# Autodesk Inventor assembly: doutai
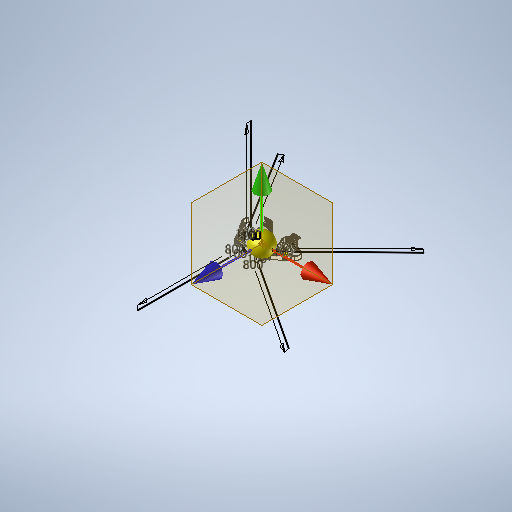
[picture p0: Inventor's stored thumbnail of the model, 512x512]
Saved by Autodesk Inventor 2025.1 (Build 291241000, 241)
## iProperties
Created: 2024-09-01
Part Number: doutai
Document SubType Name: Assembly
Designer: right
Mass: 1092.19 g
Surface Area: 3839.17 cm^2
Volume: 644.209 cm^3
Density: 1.6954 g/cm^3
Author: right
## Documents named in this file (48)
- C:\Users\right\Documents\Inventor\Vixen\doutai.iam
- C:\Users\right\Documents\Inventor\Vixen\KRS2500_scale.ipt
- C:\Users\right\Documents\Inventor\Vixen\02157_SmallDiameterHornB.ipt
- C:\Users\right\Documents\Inventor\Vixen\namida.ipt
- C:\Users\right\Documents\Inventor\Vixen\kataue.ipt
- C:\Users\right\Documents\Inventor\Vixen\kosi_v3_1.5.ipt
- C:\Users\right\Documents\Inventor\Vixen\kosipiti.ipt
- C:\Users\right\Documents\Inventor\Vixen\kosi_pti.ipt
- C:\Users\right\Documents\Inventor\Vixen\suberase.ipt
- C:\Users\right\Documents\Inventor\Vixen\kosipiti - コピー.ipt
- C:\Users\right\Documents\Inventor\Vixen\kosi_pti_MIR.ipt
- C:\Users\right\Documents\Inventor\Vixen\katasita.ipt
- C:\Users\right\Documents\Inventor\Vixen\KSHI.ipt
- C:\Users\right\Documents\Inventor\Vixen\mata3.ipt
- C:\Users\right\Documents\Inventor\Vixen\matasita.ipt
- C:\Users\right\Documents\Inventor\Vixen\kosiuke.ipt
- C:\Users\right\Documents\Inventor\Vixen\02159_SmallFreeHornC\02159_SmallFreeHornC.ipt
- C:\Users\right\Documents\Inventor\Vixen\mataroll.ipt
- C:\Users\right\Documents\Inventor\Vixen\matat3.ipt
- C:\Users\right\Documents\Inventor\Vixen\momo.ipt
- C:\Users\right\Documents\Inventor\Vixen\servolink.ipt
- C:\Users\right\Documents\Inventor\Vixen\free_link.ipt
- C:\Users\right\Documents\Inventor\Vixen\free_suzikai.ipt
- C:\Users\right\Documents\Inventor\Vixen\hiza.ipt
- C:\Users\right\Documents\Inventor\Vixen\fox.ipt
- C:\Users\right\Documents\Inventor\Vixen\mune_1.ipt
- C:\Users\right\Documents\Inventor\Vixen\mune_2.ipt
- C:\Users\right\Documents\Inventor\Vixen\badcase.ipt
- C:\Users\right\Documents\Inventor\Vixen\bad_huta.ipt
- C:\Users\right\Documents\Inventor\Vixen\450mah.ipt
- C:\Users\right\Documents\Inventor\Vixen\asikubi_asi.ipt
- C:\Users\right\Documents\Inventor\Vixen\asikubi_asi_MIR.ipt
- C:\Users\right\Documents\Inventor\Vixen\kata.ipt
- C:\Users\right\Documents\Inventor\Vixen\t3kata.ipt
- C:\Users\right\Documents\Inventor\Vixen\ude.ipt
- C:\Users\right\Documents\Inventor\V2二足Light＿仮\02159_SmallFreeHornC_MIR2.ipt
- C:\Users\right\Documents\Inventor\V2二足Light＿仮\02157_SmallDiameterHornB_MIR1.ipt
- C:\Users\right\Documents\Inventor\V2二足Light＿仮\newnewude_2.ipt
- C:\Users\right\Documents\Inventor\V2二足Light＿仮\KRS3300_scale.ipt
- C:\Users\right\Documents\Inventor\Vixen\tesaki.ipt
- C:\Users\right\Documents\Inventor\Vixen\tesaki_sukima.ipt
- C:\Users\right\Documents\Inventor\Vixen\asiura_ita.ipt
- C:\Users\right\Documents\Inventor\Vixen\ude_suzikai.ipt
- C:\Users\right\Documents\Inventor\Vixen\Long Range SHARP IR Sensors - #GP2Y0A21YK0F\Long Range SHARP IR Sensors - #GP2Y0A21YK0F\Long Range SHARP IR Sensors - #GP2Y0A21YK0F.ipt
- C:\Users\right\Documents\Inventor\Vixen\mount.ipt
- C:\Users\right\Documents\Inventor\Vixen\switch.ipt
- C:\Users\right\Documents\Inventor\Vixen\ude_sensor.ipt
- C:\Users\right\Documents\Inventor\Vixen\ude_tunagi.ipt
## Components (151 placed, 47 different names)
1. KRS2500_scale:1 — 挿入:9, 挿入:48, 挿入:49, 挿入:58, 角度:3
2. 02157_SmallDiameterHornB:2 — 挿入:9, 挿入:12, 挿入:13
3. 02157_SmallDiameterHornB:3 — 挿入:11, 挿入:23, 挿入:24
4. KRS2500_scale:2 — 挿入:11, 挿入:18, 挿入:19, 挿入:27, 挿入:28
5. kosi_v3_1.5:1 — 挿入:12, 挿入:13, 挿入:16, 挿入:17, 挿入:25, 挿入:26, フラッシュ:13, 角度:17, 角度:31
6. kosipiti:2 — 挿入:16, 挿入:17, 挿入:22, 正接:1, 正接:2, 挿入:359
7. kosi_pti:1 — 挿入:18, 挿入:19, 挿入:22, 挿入:29
8. namida:1 — 挿入:23, 挿入:24, フラッシュ:2, 挿入:126
9. suberase:1 — フラッシュ:2, 正接:1, 挿入:126, 正接:2
10. kosipiti - コピー:1 — 挿入:25, 挿入:26, 挿入:358
11. kosi_pti_MIR:1 — 挿入:27, 挿入:28, 挿入:33, 挿入:194
12. katasita:1 — 挿入:29, 挿入:33, 挿入:40, 挿入:41, 挿入:42, 挿入:43, 角度:31
13. KRS2500_scale:5 — 挿入:39, 挿入:40, 挿入:41, 挿入:44, 挿入:45, 挿入:185, 角度:22
14. KRS2500_scale:6 — 挿入:38, 挿入:42, 挿入:43, フラッシュ:7, 挿入:46, 挿入:47, 挿入:184, 角度:28
15. 02157_SmallDiameterHornB:4 — 挿入:38, 挿入:321, 挿入:322
16. 02157_SmallDiameterHornB:5 — 挿入:39, 挿入:214, 挿入:215
17. kataue:1 — フラッシュ:7, 挿入:44, 挿入:45, 挿入:46, 挿入:47, 挿入:186, 挿入:187, 挿入:188, 挿入:189, 挿入:190, 挿入:191, 挿入:379, 挿入:380
18. KSHI:1 — 挿入:48, 挿入:49, フラッシュ:8, メイト:2, メイト:4, 挿入:56
19. KRS2500_scale:7 — フラッシュ:9, メイト:2, フラッシュ:10, 挿入:50, 挿入:51, 挿入:52, 挿入:53, 挿入:61, 挿入:62, 角度:9
20. KRS2500_scale:8 — フラッシュ:8, フラッシュ:9, フラッシュ:10, メイト:4, フラッシュ:11, 挿入:54, 挿入:55, 挿入:60, 挿入:63, 角度:11, 角度:16
21. mata3:1 — フラッシュ:11, 挿入:57
22. mata3:2 — 挿入:50, 挿入:51
23. mata3:3 — 挿入:54, 挿入:55, 挿入:56, 角度:17
24. mata3:4 — 挿入:52, 挿入:53, 挿入:59
25. matasita:1 — 挿入:57, 挿入:58, 挿入:59
26. kosiuke:1 — フラッシュ:13
27. 02159_SmallFreeHornC:1 — 挿入:60, 挿入:130, 挿入:131
28. 02159_SmallFreeHornC:2 — 挿入:61, 挿入:66, 挿入:67
29. 02157_SmallDiameterHornB:6 — 挿入:62, 挿入:64, 挿入:65
30. 02157_SmallDiameterHornB:7 — 挿入:63, 挿入:132, 挿入:133
31. mataroll:1 — 挿入:64, 挿入:65, 角度:2, 挿入:68
32. mataroll:2 — 挿入:66, 挿入:67, 角度:2, 挿入:69
33. matat3:1 — 挿入:68, 挿入:69, 挿入:70, 挿入:71, 挿入:72, 挿入:73, 角度:3
34. momo:1 — 挿入:70, 挿入:71, 挿入:74, 挿入:81
35. momo:2 — 挿入:72, 挿入:73, 挿入:82
36. servolink:1 — 挿入:74, 挿入:75, 挿入:76
37. KRS2500_scale:9 — 挿入:75, 挿入:76, 挿入:77, 挿入:78, 挿入:79, 挿入:80
38. servolink:2 — 挿入:77, 挿入:78
39. 02159_SmallFreeHornC:3 — 挿入:80, 挿入:108, 挿入:109
40. 02157_SmallDiameterHornB:8 — 挿入:79, 挿入:85, 挿入:86
41. free_link:1 — 挿入:81, 角度:4, 挿入:87
42. free_link:2 — 挿入:82, 角度:4, 挿入:201, 挿入:202
43. hiza:1 — 挿入:85, 挿入:86, 挿入:87, 挿入:90, 挿入:98, 挿入:99, 角度:18
44. free_link:3 — 挿入:90, 挿入:104
45. free_link:4 — 挿入:111, 挿入:203, 挿入:204
46. momo:3 — 挿入:104, 挿入:105, 挿入:119
47. KRS2500_scale:10 — 挿入:100, 挿入:101, 挿入:102, 挿入:103
48. 02159_SmallFreeHornC:4 — 挿入:106, 挿入:107
49. 02157_SmallDiameterHornB:9 — 挿入:98, 挿入:99
50. servolink:3 — 挿入:100, 挿入:101, 挿入:110
51. servolink:4 — 挿入:102, 挿入:103, 挿入:105
52. hiza:2 — 挿入:106, 挿入:107, 挿入:108, 挿入:109
53. momo:4 — 挿入:110, 挿入:111, 挿入:118
54. mataroll:3 — 挿入:114, 挿入:115, 挿入:122, 挿入:123
55. mataroll:4 — 挿入:116, 挿入:117, 挿入:124, 挿入:125
56. matat3:2 — 挿入:114, 挿入:115, 挿入:116, 挿入:117, 挿入:118, 挿入:119
57. KRS2500_scale:11 — 角度:9, 挿入:207, 挿入:208, 挿入:209, 挿入:210
58. 02159_SmallFreeHornC:5 — 挿入:124, 挿入:125
59. 02157_SmallDiameterHornB:10 — 挿入:122, 挿入:123
60. mataroll:5 — 挿入:129, 挿入:132, 挿入:133
61. mataroll:6 — 挿入:130, 挿入:131
62. matat3:3 — 挿入:129, 角度:11, 挿入:134, 挿入:135, 挿入:136, 挿入:137
63. momo:5 — 挿入:134, 挿入:135, 挿入:352
64. momo:6 — 挿入:136, 挿入:137, 挿入:144, 挿入:147
65. KRS2500_scale:12 — 挿入:140, 挿入:141, 挿入:142, 挿入:143
66. 02159_SmallFreeHornC:6 — 挿入:152, 挿入:153
67. 02157_SmallDiameterHornB:11 — 挿入:149, 挿入:150
68. servolink:5 — 挿入:140, 挿入:141
69. servolink:6 — 挿入:142, 挿入:143, 挿入:144
70. free_link:5 — 挿入:154, 挿入:347, 挿入:348, 挿入:349, 挿入:352
71. free_link:6 — 挿入:147, 挿入:151, 挿入:350, 挿入:351
72. hiza:3 — 挿入:149, 挿入:150, 挿入:151, 挿入:157, 挿入:158, 挿入:167, 角度:26
73. hiza:4 — 挿入:152, 挿入:153, 挿入:154, 挿入:159, 挿入:346, 挿入:347
74. KRS2500_scale:13 — 挿入:160, 挿入:161, 挿入:162, 挿入:163
75. 02159_SmallFreeHornC:7 — 挿入:159
76. 02157_SmallDiameterHornB:12 — 挿入:157, 挿入:158
77. servolink:7 — 挿入:160, 挿入:161, 挿入:176
78. servolink:8 — 挿入:162, 挿入:163
79. free_link:7 — 挿入:179, 挿入:197, 挿入:198, 挿入:346
80. free_link:8 — 挿入:167, 挿入:199, 挿入:200
81. momo:7 — 挿入:178, 挿入:179
82. momo:8 — 挿入:176, 挿入:177
83. mataroll:7 — 挿入:182, 挿入:183
84. mataroll:8
85. matat3:4 — 挿入:177, 挿入:178
86. KRS2500_scale:14 — 角度:16, フラッシュ:17, 挿入:205, 挿入:206, 挿入:288, 挿入:289
87. 02159_SmallFreeHornC:8
88. 02157_SmallDiameterHornB:13 — 挿入:182, 挿入:183
89. 02159_SmallFreeHornC:9 — 挿入:184, 挿入:323
90. 02159_SmallFreeHornC:10 — 挿入:185, 挿入:216, 挿入:217
91. fox:1 — 挿入:186, 挿入:187
92. mune_1:1 — 挿入:188, 挿入:189
93. mune_2:1 — 挿入:190, 挿入:191, メイト:8, メイト:9, メイト:10, 挿入:377, 挿入:378
94. badcase:1 — フラッシュ:16, 挿入:192, 挿入:193, メイト:5, 挿入:194
95. bad_huta:1 — フラッシュ:16, 挿入:192, 挿入:193, メイト:6, 正接:3
96. 450mah:1 — メイト:5, メイト:6, 正接:3
97. free_suzikai:1 — 挿入:203, 挿入:204, 角度:19
98. free_suzikai:2 — 挿入:201, 挿入:202, 角度:18, 角度:19
99. free_suzikai:4 — 挿入:197, 挿入:198, 挿入:199, 挿入:200, 角度:27
100. asikubi_asi:1 — フラッシュ:17, メイト:7, フラッシュ:18, 挿入:288, 挿入:289
101. asikubi_asi:2 — 挿入:205, 挿入:206, フラッシュ:19
102. asikubi_asi_MIR:1 — 挿入:207, 挿入:208, 挿入:292
103. asikubi_asi_MIR:2 — 挿入:209, 挿入:210, 挿入:290, 挿入:291
104. kata:1 — 挿入:214, 挿入:215, 挿入:218, 挿入:219
105. kata:2 — 挿入:216, 挿入:217, 挿入:220, 挿入:221
106. t3kata:1 — 挿入:218, 挿入:219, 挿入:220, 挿入:221, 挿入:222, 挿入:223, 挿入:224, 挿入:225, 角度:22
107. kata:3 — 挿入:222, 挿入:223, 挿入:230, 挿入:231
108. kata:4 — 挿入:224, 挿入:225, 挿入:228, 挿入:229
109. KRS2500_scale:15 — 挿入:337, 挿入:338, 挿入:363
110. 02157_SmallDiameterHornB:14 — 挿入:228, 挿入:229
111. 02159_SmallFreeHornC:11 — 挿入:230, 挿入:231
112. 02159_SmallFreeHornC_MIR2:1 — 挿入:242, 挿入:243, 挿入:295
113. 02157_SmallDiameterHornB_MIR1:1 — 挿入:246, 挿入:339, 挿入:340
114. newnewude_2:1 — 挿入:242, 挿入:243, 挿入:342
115. KRS3300_scale:1 — 挿入:246, フラッシュ:20, 挿入:293, 挿入:294, 挿入:295, 挿入:355
116. asiura_ita:1 — メイト:7, フラッシュ:18, フラッシュ:19
117. asiura_ita:2 — 挿入:290, 挿入:291, 挿入:292
118. tesaki:1 — フラッシュ:20, 挿入:334, 挿入:341, 挿入:355
119. tesaki:2 — 挿入:293, 挿入:294, フラッシュ:21, 挿入:333, 挿入:354
120. tesaki_sukima:1 — フラッシュ:21, 挿入:333, 挿入:334, 挿入:341, 挿入:354
121. ude:1 — フラッシュ:25, 挿入:335, 挿入:336, 挿入:337, 挿入:338, 挿入:339, 挿入:340, メイト:11, 挿入:366, 挿入:368
122. ude_suzikai:1 — フラッシュ:25, 挿入:335, 挿入:336, 挿入:342, 角度:30, メイト:12, フラッシュ:32, 挿入:362, 挿入:364
123. kata:9 — 挿入:321, 挿入:322
124. kata:10 — 挿入:323
125. t3kata:3 — 角度:28
126. kata:11
127. kata:12
128. KRS2500_scale:17 — 挿入:324, 挿入:325, 挿入:373, 挿入:374
129. 02157_SmallDiameterHornB:16
130. 02159_SmallFreeHornC:13
131. 02159_SmallFreeHornC_MIR2:3
132. 02157_SmallDiameterHornB_MIR1:3 — 挿入:317, 挿入:318
133. newnewude_2:3 — 挿入:353
134. KRS3300_scale:3 — 挿入:330, 挿入:331
135. tesaki:4 — 挿入:328, 挿入:329
136. tesaki_sukima:2 — 挿入:328, 挿入:329, 挿入:332
137. ude:2 — 挿入:316, 挿入:317, 挿入:318, 挿入:319, 挿入:320, 挿入:324, 挿入:325, 挿入:376
138. ude_suzikai:2 — 挿入:316, 挿入:319, 挿入:320, 挿入:353, 挿入:375
139. tesaki:5 — 挿入:330, 挿入:331, 挿入:332
140. free_suzikai:5 — 挿入:348, 挿入:349, 挿入:350, 挿入:351, 角度:26, 角度:27
141. Long Range SHARP IR Sensors - #GP2Y0A21YK0F:1 — 挿入:356, 挿入:357
142. mount:1 — 挿入:356, 挿入:357, 挿入:358, 挿入:359
143. switch:1 — メイト:8, メイト:9, メイト:10
144. Long Range SHARP IR Sensors - #GP2Y0A21YK0F:2 — 角度:30, 挿入:360, 挿入:361
145. ude_sensor:1 — 挿入:360, 挿入:361, メイト:11, メイト:12, 挿入:365, 挿入:366, 挿入:367, 挿入:368
146. ude_tunagi:1 — フラッシュ:32, 挿入:362, 挿入:363, 挿入:364, 挿入:365, 挿入:367
147. Long Range SHARP IR Sensors - #GP2Y0A21YK0F:3
148. ude_sensor:2 — 挿入:376
149. ude_tunagi:2 — 挿入:373, 挿入:374, 挿入:375
150. Long Range SHARP IR Sensors - #GP2Y0A21YK0F:4 — 挿入:377, 挿入:378
151. Long Range SHARP IR Sensors - #GP2Y0A21YK0F:5 — 挿入:379, 挿入:380
## Relationships (334: Insert 282, Angle 20, Flush 19, Mate 10, Tangent 3)
- 挿入:9 [Insert]: KRS2500_scale:1 ↔ 02157_SmallDiameterHornB:2
- 挿入:11 [Insert]: 02157_SmallDiameterHornB:3 ↔ KRS2500_scale:2
- 挿入:12 [Insert]: 02157_SmallDiameterHornB:2 ↔ kosi_v3_1.5:1
- 挿入:13 [Insert]: 02157_SmallDiameterHornB:2 ↔ kosi_v3_1.5:1
- 挿入:16 [Insert]: kosi_v3_1.5:1 ↔ kosipiti:2
- 挿入:17 [Insert]: kosi_v3_1.5:1 ↔ kosipiti:2
- 挿入:18 [Insert]: KRS2500_scale:2 ↔ kosi_pti:1
- 挿入:19 [Insert]: KRS2500_scale:2 ↔ kosi_pti:1
- 挿入:22 [Insert] (5.5 mm): kosipiti:2 ↔ kosi_pti:1
- 挿入:23 [Insert]: 02157_SmallDiameterHornB:3 ↔ namida:1
- 挿入:24 [Insert]: 02157_SmallDiameterHornB:3 ↔ namida:1
- フラッシュ:2 [Flush]: namida:1 ↔ suberase:1
- 挿入:25 [Insert]: kosi_v3_1.5:1 ↔ kosipiti - コピー:1
- 挿入:26 [Insert]: kosi_v3_1.5:1 ↔ kosipiti - コピー:1
- 挿入:27 [Insert]: KRS2500_scale:2 ↔ kosi_pti_MIR:1
- 挿入:28 [Insert]: KRS2500_scale:2 ↔ kosi_pti_MIR:1
- 挿入:29 [Insert]: kosi_pti:1 ↔ katasita:1
- 挿入:33 [Insert]: kosi_pti_MIR:1 ↔ katasita:1
- 挿入:38 [Insert]: KRS2500_scale:6 ↔ 02157_SmallDiameterHornB:4
- 挿入:39 [Insert]: KRS2500_scale:5 ↔ 02157_SmallDiameterHornB:5
- 挿入:40 [Insert]: katasita:1 ↔ KRS2500_scale:5
- 挿入:41 [Insert]: katasita:1 ↔ KRS2500_scale:5
- 挿入:42 [Insert]: katasita:1 ↔ KRS2500_scale:6
- 挿入:43 [Insert]: katasita:1 ↔ KRS2500_scale:6
- フラッシュ:7 [Flush]: KRS2500_scale:6 ↔ kataue:1
- 挿入:44 [Insert]: KRS2500_scale:5 ↔ kataue:1
- 挿入:45 [Insert]: KRS2500_scale:5 ↔ kataue:1
- 挿入:46 [Insert]: KRS2500_scale:6 ↔ kataue:1
- 挿入:47 [Insert]: KRS2500_scale:6 ↔ kataue:1
- 正接:1 [Tangent]: kosipiti:2 ↔ suberase:1
- 挿入:48 [Insert]: KRS2500_scale:1 ↔ KSHI:1
- 挿入:49 [Insert]: KRS2500_scale:1 ↔ KSHI:1
- フラッシュ:8 [Flush]: KSHI:1 ↔ KRS2500_scale:8
- フラッシュ:9 [Flush]: KRS2500_scale:7 ↔ KRS2500_scale:8
- メイト:2 [Mate]: KSHI:1 ↔ KRS2500_scale:7
- フラッシュ:10 [Flush]: KRS2500_scale:7 ↔ KRS2500_scale:8
- メイト:4 [Mate]: KSHI:1 ↔ KRS2500_scale:8
- フラッシュ:11 [Flush]: KRS2500_scale:8 ↔ mata3:1
- 挿入:50 [Insert]: KRS2500_scale:7 ↔ mata3:2
- 挿入:51 [Insert]: KRS2500_scale:7 ↔ mata3:2
- 挿入:52 [Insert]: KRS2500_scale:7 ↔ mata3:4
- 挿入:53 [Insert]: KRS2500_scale:7 ↔ mata3:4
- 挿入:54 [Insert]: KRS2500_scale:8 ↔ mata3:3
- 挿入:55 [Insert]: KRS2500_scale:8 ↔ mata3:3
- 挿入:56 [Insert]: KSHI:1 ↔ mata3:3
- 挿入:57 [Insert]: mata3:1 ↔ matasita:1
- 挿入:58 [Insert]: KRS2500_scale:1 ↔ matasita:1
- 挿入:59 [Insert]: mata3:4 ↔ matasita:1
- フラッシュ:13 [Flush]: kosi_v3_1.5:1 ↔ kosiuke:1
- 挿入:60 [Insert]: KRS2500_scale:8 ↔ 02159_SmallFreeHornC:1
- 挿入:61 [Insert]: KRS2500_scale:7 ↔ 02159_SmallFreeHornC:2
- 挿入:62 [Insert]: KRS2500_scale:7 ↔ 02157_SmallDiameterHornB:6
- 挿入:63 [Insert]: KRS2500_scale:8 ↔ 02157_SmallDiameterHornB:7
- 挿入:64 [Insert]: 02157_SmallDiameterHornB:6 ↔ mataroll:1
- 挿入:65 [Insert]: 02157_SmallDiameterHornB:6 ↔ mataroll:1
- 挿入:66 [Insert]: 02159_SmallFreeHornC:2 ↔ mataroll:2
- 挿入:67 [Insert]: 02159_SmallFreeHornC:2 ↔ mataroll:2
- 角度:2 [Angle] (0 deg): mataroll:1 ↔ mataroll:2
- 挿入:68 [Insert]: mataroll:1 ↔ matat3:1
- 挿入:69 [Insert]: mataroll:2 ↔ matat3:1
- 挿入:70 [Insert]: matat3:1 ↔ momo:1
- 挿入:71 [Insert]: matat3:1 ↔ momo:1
- 挿入:72 [Insert]: matat3:1 ↔ momo:2
- 挿入:73 [Insert]: matat3:1 ↔ momo:2
- 挿入:74 [Insert] (3 mm): momo:1 ↔ servolink:1
- 挿入:75 [Insert]: servolink:1 ↔ KRS2500_scale:9
- 挿入:76 [Insert]: servolink:1 ↔ KRS2500_scale:9
- 挿入:77 [Insert]: KRS2500_scale:9 ↔ servolink:2
- 挿入:78 [Insert]: KRS2500_scale:9 ↔ servolink:2
- 挿入:79 [Insert]: KRS2500_scale:9 ↔ 02157_SmallDiameterHornB:8
- 挿入:80 [Insert]: KRS2500_scale:9 ↔ 02159_SmallFreeHornC:3
- 角度:3 [Angle] (15 deg): KRS2500_scale:1 ↔ matat3:1
- 挿入:81 [Insert] (3 mm): momo:1 ↔ free_link:1
- 挿入:82 [Insert] (3 mm): momo:2 ↔ free_link:2
- 角度:4 [Angle] (0 deg): free_link:1 ↔ free_link:2
- 挿入:85 [Insert]: 02157_SmallDiameterHornB:8 ↔ hiza:1
- 挿入:86 [Insert]: 02157_SmallDiameterHornB:8 ↔ hiza:1
- 挿入:87 [Insert] (3 mm): free_link:1 ↔ hiza:1
- [Angle] (0 deg): free_link:3 ↔ free_link:4
- 挿入:90 [Insert] (3 mm): hiza:1 ↔ free_link:3
- [Insert]: KRS2500_scale:10 ↔ 02157_SmallDiameterHornB:9
- [Insert]: KRS2500_scale:10 ↔ 02159_SmallFreeHornC:4
- 挿入:98 [Insert]: hiza:1 ↔ 02157_SmallDiameterHornB:9
- 挿入:99 [Insert]: hiza:1 ↔ 02157_SmallDiameterHornB:9
- 挿入:100 [Insert]: KRS2500_scale:10 ↔ servolink:3
- 挿入:101 [Insert]: KRS2500_scale:10 ↔ servolink:3
- 挿入:102 [Insert]: KRS2500_scale:10 ↔ servolink:4
- 挿入:103 [Insert]: KRS2500_scale:10 ↔ servolink:4
- 挿入:104 [Insert] (3 mm): free_link:3 ↔ momo:3
- 挿入:105 [Insert] (3 mm): momo:3 ↔ servolink:4
- 挿入:106 [Insert]: 02159_SmallFreeHornC:4 ↔ hiza:2
- 挿入:107 [Insert]: 02159_SmallFreeHornC:4 ↔ hiza:2
- 挿入:108 [Insert]: 02159_SmallFreeHornC:3 ↔ hiza:2
- 挿入:109 [Insert]: 02159_SmallFreeHornC:3 ↔ hiza:2
- 挿入:110 [Insert] (3 mm): servolink:3 ↔ momo:4
- 挿入:111 [Insert] (3 mm): free_link:4 ↔ momo:4
- [Angle] (0 deg): mataroll:3 ↔ mataroll:4
- [Insert]: mataroll:3 ↔ matat3:2
- [Insert]: mataroll:4 ↔ matat3:2
- 挿入:114 [Insert]: mataroll:3 ↔ matat3:2
- 挿入:115 [Insert]: mataroll:3 ↔ matat3:2
- 挿入:116 [Insert]: mataroll:4 ↔ matat3:2
- 挿入:117 [Insert]: mataroll:4 ↔ matat3:2
- 挿入:118 [Insert]: momo:4 ↔ matat3:2
- 挿入:119 [Insert]: momo:3 ↔ matat3:2
- [Insert]: KRS2500_scale:11 ↔ 02157_SmallDiameterHornB:10
- [Insert]: KRS2500_scale:11 ↔ 02159_SmallFreeHornC:5
- 挿入:122 [Insert]: mataroll:3 ↔ 02157_SmallDiameterHornB:10
- 挿入:123 [Insert]: mataroll:3 ↔ 02157_SmallDiameterHornB:10
- 挿入:124 [Insert]: mataroll:4 ↔ 02159_SmallFreeHornC:5
- 挿入:125 [Insert]: mataroll:4 ↔ 02159_SmallFreeHornC:5
- 挿入:126 [Insert]: namida:1 ↔ suberase:1
- 正接:2 [Tangent]: kosipiti:2 ↔ suberase:1
- 角度:9 [Angle] (0 deg): KRS2500_scale:7 ↔ KRS2500_scale:11
- [Angle] (0 deg): mataroll:5 ↔ mataroll:6
- [Insert]: mataroll:5 ↔ matat3:3
- [Insert]: mataroll:6 ↔ matat3:3
- 挿入:129 [Insert]: mataroll:5 ↔ matat3:3
- 挿入:130 [Insert]: 02159_SmallFreeHornC:1 ↔ mataroll:6
- 挿入:131 [Insert]: 02159_SmallFreeHornC:1 ↔ mataroll:6
- 挿入:132 [Insert]: 02157_SmallDiameterHornB:7 ↔ mataroll:5
- 挿入:133 [Insert]: 02157_SmallDiameterHornB:7 ↔ mataroll:5
- 角度:11 [Angle] (15 deg): KRS2500_scale:8 ↔ matat3:3
- 挿入:134 [Insert]: matat3:3 ↔ momo:5
- 挿入:135 [Insert]: matat3:3 ↔ momo:5
- 挿入:136 [Insert]: matat3:3 ↔ momo:6
- 挿入:137 [Insert]: matat3:3 ↔ momo:6
- [Insert]: KRS2500_scale:12 ↔ 02157_SmallDiameterHornB:11
- [Insert]: KRS2500_scale:12 ↔ 02159_SmallFreeHornC:6
- 挿入:140 [Insert]: KRS2500_scale:12 ↔ servolink:5
- 挿入:141 [Insert]: KRS2500_scale:12 ↔ servolink:5
- 挿入:142 [Insert]: KRS2500_scale:12 ↔ servolink:6
- 挿入:143 [Insert]: KRS2500_scale:12 ↔ servolink:6
- 挿入:144 [Insert] (3 mm): momo:6 ↔ servolink:6
- 挿入:147 [Insert] (3 mm): momo:6 ↔ free_link:6
- 挿入:149 [Insert]: 02157_SmallDiameterHornB:11 ↔ hiza:3
- 挿入:150 [Insert]: 02157_SmallDiameterHornB:11 ↔ hiza:3
- 挿入:151 [Insert] (3 mm): free_link:6 ↔ hiza:3
- 挿入:152 [Insert]: 02159_SmallFreeHornC:6 ↔ hiza:4
- 挿入:153 [Insert]: 02159_SmallFreeHornC:6 ↔ hiza:4
- 挿入:154 [Insert] (3 mm): free_link:5 ↔ hiza:4
- [Insert]: KRS2500_scale:13 ↔ 02157_SmallDiameterHornB:12
- [Insert]: KRS2500_scale:13 ↔ 02159_SmallFreeHornC:7
- 挿入:157 [Insert]: hiza:3 ↔ 02157_SmallDiameterHornB:12
- 挿入:158 [Insert]: hiza:3 ↔ 02157_SmallDiameterHornB:12
- 挿入:159 [Insert]: hiza:4 ↔ 02159_SmallFreeHornC:7
- 挿入:160 [Insert]: KRS2500_scale:13 ↔ servolink:7
- 挿入:161 [Insert]: KRS2500_scale:13 ↔ servolink:7
- 挿入:162 [Insert]: KRS2500_scale:13 ↔ servolink:8
- 挿入:163 [Insert]: KRS2500_scale:13 ↔ servolink:8
- [Angle] (0 deg): free_link:7 ↔ free_link:8
- 挿入:167 [Insert] (3 mm): hiza:3 ↔ free_link:8
- [Angle] (0 deg): mataroll:7 ↔ mataroll:8
- [Insert]: mataroll:7 ↔ matat3:4
- [Insert]: mataroll:8 ↔ matat3:4
- [Insert]: mataroll:7 ↔ matat3:4
- [Insert]: mataroll:7 ↔ matat3:4
- [Insert]: mataroll:8 ↔ matat3:4
- [Insert]: mataroll:8 ↔ matat3:4
- [Insert]: momo:8 ↔ matat3:4
- [Insert]: momo:7 ↔ matat3:4
- 挿入:176 [Insert] (3 mm): servolink:7 ↔ momo:8
- 挿入:177 [Insert]: momo:8 ↔ matat3:4
- 挿入:178 [Insert]: momo:7 ↔ matat3:4
- 挿入:179 [Insert] (3 mm): free_link:7 ↔ momo:7
- [Insert]: KRS2500_scale:14 ↔ 02157_SmallDiameterHornB:13
- [Insert]: KRS2500_scale:14 ↔ 02159_SmallFreeHornC:8
- 挿入:182 [Insert]: mataroll:7 ↔ 02157_SmallDiameterHornB:13
- 挿入:183 [Insert]: mataroll:7 ↔ 02157_SmallDiameterHornB:13
- 角度:16 [Angle] (0 deg): KRS2500_scale:8 ↔ KRS2500_scale:14
- 角度:17 [Angle] (0 deg): kosi_v3_1.5:1 ↔ mata3:3
- 挿入:184 [Insert]: KRS2500_scale:6 ↔ 02159_SmallFreeHornC:9
- 挿入:185 [Insert]: KRS2500_scale:5 ↔ 02159_SmallFreeHornC:10
- 挿入:186 [Insert]: kataue:1 ↔ fox:1
- 挿入:187 [Insert]: kataue:1 ↔ fox:1
- 挿入:188 [Insert]: kataue:1 ↔ mune_1:1
- 挿入:189 [Insert]: kataue:1 ↔ mune_1:1
- 挿入:190 [Insert]: kataue:1 ↔ mune_2:1
- 挿入:191 [Insert]: kataue:1 ↔ mune_2:1
- フラッシュ:16 [Flush]: badcase:1 ↔ bad_huta:1
- 挿入:192 [Insert]: badcase:1 ↔ bad_huta:1
- 挿入:193 [Insert]: badcase:1 ↔ bad_huta:1
- メイト:5 [Mate]: badcase:1 ↔ 450mah:1
- 挿入:194 [Insert] (1 mm): kosi_pti_MIR:1 ↔ badcase:1
- メイト:6 [Mate]: bad_huta:1 ↔ 450mah:1
- 正接:3 [Tangent]: bad_huta:1 ↔ 450mah:1
- 挿入:197 [Insert]: free_link:7 ↔ free_suzikai:4
- 挿入:198 [Insert]: free_link:7 ↔ free_suzikai:4
- 挿入:199 [Insert]: free_link:8 ↔ free_suzikai:4
- 挿入:200 [Insert]: free_link:8 ↔ free_suzikai:4
- 挿入:201 [Insert]: free_link:2 ↔ free_suzikai:2
- 挿入:202 [Insert]: free_link:2 ↔ free_suzikai:2
- 挿入:203 [Insert]: free_link:4 ↔ free_suzikai:1
- 挿入:204 [Insert]: free_link:4 ↔ free_suzikai:1
- 角度:18 [Angle] (40 deg): hiza:1 ↔ free_suzikai:2
- 角度:19 [Angle] (-80 deg): free_suzikai:1 ↔ free_suzikai:2
- フラッシュ:17 [Flush]: KRS2500_scale:14 ↔ asikubi_asi:1
- 挿入:205 [Insert]: KRS2500_scale:14 ↔ asikubi_asi:2
- 挿入:206 [Insert]: KRS2500_scale:14 ↔ asikubi_asi:2
- 挿入:207 [Insert]: KRS2500_scale:11 ↔ asikubi_asi_MIR:1
- 挿入:208 [Insert]: KRS2500_scale:11 ↔ asikubi_asi_MIR:1
- 挿入:209 [Insert]: KRS2500_scale:11 ↔ asikubi_asi_MIR:2
- 挿入:210 [Insert]: KRS2500_scale:11 ↔ asikubi_asi_MIR:2
- 挿入:214 [Insert]: 02157_SmallDiameterHornB:5 ↔ kata:1
- 挿入:215 [Insert]: 02157_SmallDiameterHornB:5 ↔ kata:1
- 挿入:216 [Insert]: 02159_SmallFreeHornC:10 ↔ kata:2
- 挿入:217 [Insert]: 02159_SmallFreeHornC:10 ↔ kata:2
- 挿入:218 [Insert]: kata:1 ↔ t3kata:1
- 挿入:219 [Insert]: kata:1 ↔ t3kata:1
- 挿入:220 [Insert]: kata:2 ↔ t3kata:1
- 挿入:221 [Insert]: kata:2 ↔ t3kata:1
- 挿入:222 [Insert]: t3kata:1 ↔ kata:3
- 挿入:223 [Insert]: t3kata:1 ↔ kata:3
- 挿入:224 [Insert]: t3kata:1 ↔ kata:4
- 挿入:225 [Insert]: t3kata:1 ↔ kata:4
- [Insert]: KRS2500_scale:15 ↔ 02157_SmallDiameterHornB:14
- [Insert]: KRS2500_scale:15 ↔ 02159_SmallFreeHornC:11
- 挿入:228 [Insert]: kata:4 ↔ 02157_SmallDiameterHornB:14
- 挿入:229 [Insert]: kata:4 ↔ 02157_SmallDiameterHornB:14
- 挿入:230 [Insert]: kata:3 ↔ 02159_SmallFreeHornC:11
- 挿入:231 [Insert]: kata:3 ↔ 02159_SmallFreeHornC:11
- 角度:22 [Angle] (0 deg): KRS2500_scale:5 ↔ t3kata:1
- 挿入:242 [Insert]: 02159_SmallFreeHornC_MIR2:1 ↔ newnewude_2:1
- 挿入:243 [Insert]: 02159_SmallFreeHornC_MIR2:1 ↔ newnewude_2:1
- 挿入:246 [Insert]: 02157_SmallDiameterHornB_MIR1:1 ↔ KRS3300_scale:1
- メイト:7 [Mate]: asikubi_asi:1 ↔ asiura_ita:1
- フラッシュ:18 [Flush] (-3 mm): asikubi_asi:1 ↔ asiura_ita:1
- 挿入:288 [Insert]: KRS2500_scale:14 ↔ asikubi_asi:1
- 挿入:289 [Insert]: KRS2500_scale:14 ↔ asikubi_asi:1
- フラッシュ:19 [Flush] (15 mm): asikubi_asi:2 ↔ asiura_ita:1
- 挿入:290 [Insert]: asikubi_asi_MIR:2 ↔ asiura_ita:2
- 挿入:291 [Insert]: asikubi_asi_MIR:2 ↔ asiura_ita:2
- 挿入:292 [Insert]: asikubi_asi_MIR:1 ↔ asiura_ita:2
- フラッシュ:20 [Flush]: KRS3300_scale:1 ↔ tesaki:1
- 挿入:293 [Insert]: KRS3300_scale:1 ↔ tesaki:2
- 挿入:294 [Insert]: KRS3300_scale:1 ↔ tesaki:2
- 挿入:295 [Insert]: 02159_SmallFreeHornC_MIR2:1 ↔ KRS3300_scale:1
- フラッシュ:21 [Flush]: tesaki:2 ↔ tesaki_sukima:1
- フラッシュ:25 [Flush]: ude:1 ↔ ude_suzikai:1
- [Insert]: kata:9 ↔ t3kata:3
- [Insert]: kata:9 ↔ t3kata:3
- [Insert]: kata:10 ↔ t3kata:3
- [Insert]: kata:10 ↔ t3kata:3
- [Insert]: t3kata:3 ↔ kata:11
- [Insert]: t3kata:3 ↔ kata:11
- [Insert]: t3kata:3 ↔ kata:12
- [Insert]: t3kata:3 ↔ kata:12
- [Insert]: KRS2500_scale:17 ↔ 02157_SmallDiameterHornB:16
- [Insert]: KRS2500_scale:17 ↔ 02159_SmallFreeHornC:13
- [Insert]: kata:12 ↔ 02157_SmallDiameterHornB:16
- [Insert]: kata:12 ↔ 02157_SmallDiameterHornB:16
- [Insert]: kata:11 ↔ 02159_SmallFreeHornC:13
- [Insert]: kata:11 ↔ 02159_SmallFreeHornC:13
- [Insert]: 02159_SmallFreeHornC_MIR2:3 ↔ newnewude_2:3
- [Insert]: 02159_SmallFreeHornC_MIR2:3 ↔ newnewude_2:3
- [Insert]: 02157_SmallDiameterHornB_MIR1:3 ↔ KRS3300_scale:3
- [Insert]: KRS3300_scale:3 ↔ tesaki:4
- [Insert]: KRS3300_scale:3 ↔ tesaki:4
- [Insert]: 02159_SmallFreeHornC_MIR2:3 ↔ KRS3300_scale:3
- [Flush]: tesaki:4 ↔ tesaki_sukima:2
- [Flush]: KRS2500_scale:17 ↔ 02157_SmallDiameterHornB_MIR1:3
- [Flush]: KRS2500_scale:17 ↔ ude:2
- [Flush]: ude:2 ↔ ude_suzikai:2
- 挿入:316 [Insert]: ude:2 ↔ ude_suzikai:2
- 挿入:317 [Insert]: 02157_SmallDiameterHornB_MIR1:3 ↔ ude:2
- 挿入:318 [Insert]: 02157_SmallDiameterHornB_MIR1:3 ↔ ude:2
- 挿入:319 [Insert]: ude:2 ↔ ude_suzikai:2
- 挿入:320 [Insert]: ude:2 ↔ ude_suzikai:2
- 挿入:321 [Insert]: 02157_SmallDiameterHornB:4 ↔ kata:9
- 挿入:322 [Insert]: 02157_SmallDiameterHornB:4 ↔ kata:9
- 挿入:323 [Insert]: 02159_SmallFreeHornC:9 ↔ kata:10
- 挿入:324 [Insert]: KRS2500_scale:17 ↔ ude:2
- 挿入:325 [Insert]: KRS2500_scale:17 ↔ ude:2
- 挿入:328 [Insert]: tesaki:4 ↔ tesaki_sukima:2
- 挿入:329 [Insert]: tesaki:4 ↔ tesaki_sukima:2
- 挿入:330 [Insert]: KRS3300_scale:3 ↔ tesaki:5
- 挿入:331 [Insert]: KRS3300_scale:3 ↔ tesaki:5
- 挿入:332 [Insert]: tesaki_sukima:2 ↔ tesaki:5
- 挿入:333 [Insert]: tesaki:2 ↔ tesaki_sukima:1
- 挿入:334 [Insert]: tesaki:1 ↔ tesaki_sukima:1
- 挿入:335 [Insert]: ude:1 ↔ ude_suzikai:1
- 挿入:336 [Insert]: ude:1 ↔ ude_suzikai:1
- 挿入:337 [Insert]: KRS2500_scale:15 ↔ ude:1
- 挿入:338 [Insert]: KRS2500_scale:15 ↔ ude:1
- 挿入:339 [Insert]: 02157_SmallDiameterHornB_MIR1:1 ↔ ude:1
- 挿入:340 [Insert]: 02157_SmallDiameterHornB_MIR1:1 ↔ ude:1
- 挿入:341 [Insert]: tesaki:1 ↔ tesaki_sukima:1
- 挿入:342 [Insert]: newnewude_2:1 ↔ ude_suzikai:1
- 挿入:346 [Insert] (3 mm): hiza:4 ↔ free_link:7
- 挿入:347 [Insert] (3 mm): free_link:5 ↔ hiza:4
- 挿入:348 [Insert]: free_link:5 ↔ free_suzikai:5
- 挿入:349 [Insert]: free_link:5 ↔ free_suzikai:5
- 挿入:350 [Insert]: free_link:6 ↔ free_suzikai:5
- 挿入:351 [Insert]: free_link:6 ↔ free_suzikai:5
- 挿入:352 [Insert] (3 mm): momo:5 ↔ free_link:5
- 角度:26 [Angle] (-40 deg): hiza:3 ↔ free_suzikai:5
- 角度:27 [Angle] (80 deg): free_suzikai:4 ↔ free_suzikai:5
- 挿入:353 [Insert]: newnewude_2:3 ↔ ude_suzikai:2
- 角度:28 [Angle] (0 deg): KRS2500_scale:6 ↔ t3kata:3
- 挿入:354 [Insert]: tesaki:2 ↔ tesaki_sukima:1
- 挿入:355 [Insert]: KRS3300_scale:1 ↔ tesaki:1
- 挿入:356 [Insert]: Long Range SHARP IR Sensors - #GP2Y0A21YK0F:1 ↔ mount:1
- 挿入:357 [Insert]: Long Range SHARP IR Sensors - #GP2Y0A21YK0F:1 ↔ mount:1
- メイト:8 [Mate]: mune_2:1 ↔ switch:1
- メイト:9 [Mate]: mune_2:1 ↔ switch:1
- メイト:10 [Mate]: mune_2:1 ↔ switch:1
- 挿入:358 [Insert]: kosipiti - コピー:1 ↔ mount:1
- 挿入:359 [Insert]: kosipiti:2 ↔ mount:1
- 角度:30 [Angle] (0 deg): ude_suzikai:1 ↔ Long Range SHARP IR Sensors - #GP2Y0A21YK0F:2
- 挿入:360 [Insert]: Long Range SHARP IR Sensors - #GP2Y0A21YK0F:2 ↔ ude_sensor:1
- 挿入:361 [Insert]: Long Range SHARP IR Sensors - #GP2Y0A21YK0F:2 ↔ ude_sensor:1
- メイト:11 [Mate]: ude:1 ↔ ude_sensor:1
- メイト:12 [Mate]: ude_suzikai:1 ↔ ude_sensor:1
- フラッシュ:32 [Flush]: ude_suzikai:1 ↔ ude_tunagi:1
- 挿入:362 [Insert]: ude_suzikai:1 ↔ ude_tunagi:1
- 挿入:363 [Insert]: KRS2500_scale:15 ↔ ude_tunagi:1
- 挿入:364 [Insert]: ude_suzikai:1 ↔ ude_tunagi:1
- 挿入:365 [Insert]: ude_sensor:1 ↔ ude_tunagi:1
- 挿入:366 [Insert]: ude:1 ↔ ude_sensor:1
- 挿入:367 [Insert]: ude_sensor:1 ↔ ude_tunagi:1
- 挿入:368 [Insert]: ude:1 ↔ ude_sensor:1
- [Insert]: Long Range SHARP IR Sensors - #GP2Y0A21YK0F:3 ↔ ude_sensor:2
- [Insert]: Long Range SHARP IR Sensors - #GP2Y0A21YK0F:3 ↔ ude_sensor:2
- [Insert]: ude_sensor:2 ↔ ude_tunagi:2
- [Insert]: ude_sensor:2 ↔ ude_tunagi:2
- 挿入:373 [Insert]: KRS2500_scale:17 ↔ ude_tunagi:2
- 挿入:374 [Insert]: KRS2500_scale:17 ↔ ude_tunagi:2
- 挿入:375 [Insert]: ude_suzikai:2 ↔ ude_tunagi:2
- 挿入:376 [Insert]: ude:2 ↔ ude_sensor:2
- 角度:31 [Angle] (0 deg): kosi_v3_1.5:1 ↔ katasita:1
- 挿入:377 [Insert]: mune_2:1 ↔ Long Range SHARP IR Sensors - #GP2Y0A21YK0F:4
- 挿入:378 [Insert]: mune_2:1 ↔ Long Range SHARP IR Sensors - #GP2Y0A21YK0F:4
- 挿入:379 [Insert]: kataue:1 ↔ Long Range SHARP IR Sensors - #GP2Y0A21YK0F:5
- 挿入:380 [Insert]: kataue:1 ↔ Long Range SHARP IR Sensors - #GP2Y0A21YK0F:5
## Named parameters: d170_d163 = 0 deg, d178_d158 = 0 mm, d179_d159 = 0 mm, d195_d148 = 0 mm, d196_d146 = 0 deg, d197_d147 = 0 mm, d204_d178_d158 = 0 mm, d205_d179_d159 = 0 mm, d215_d148 = 0 mm, d216_d146 = 0 deg, d217_d147 = 0 mm, d228_d158 = 0 mm, d229_d159 = 0 mm, d247_d178_d158 = 0 mm, d248_d179_d159 = 0 mm, d261_d236_d163 = 0 deg, d265_d198 = 0 mm, d266_d199 = 0 mm, d267_d200 = 0 mm, d268_d201 = 0 mm, d269_d202 = 0 mm, d270_d203 = 0 mm, d271_d195_d148 = 0 mm, d272_d196_d146 = 0 deg, d273_d197_d147 = 0 mm, d278_d204_d178_d158 = 0 mm, d279_d205_d179_d159 = 0 mm, d342_d285 = 0 mm, d343_d103 = 0 mm, d444_d344 = 0 mm, d445_d345 = 0 mm, d446_d346 = 0 mm, d447_d347 = 0 mm, d449_d334 = 0 mm, d450_d335 = 0 mm, d451_d336 = 0 mm, d452_d337 = 0 mm, d453_d338 = 0 mm, d454_d339 = 0 mm, d455_d340 = 0 mm, d456_d341 = 0 mm, d457_d342_d285 = 0 mm, d458_d343_d103 = 0 mm, d459_d370 = 0 mm, d460_d371 = 0 mm, d461_d374 = 0 mm, d464_d435 = 0 mm, d465_d436 = 0 mm, d466_d437 = 0 mm, d467_d438 = 0 mm, d469_d440 = 0 mm, d471_d442 = 0 mm, d472_d443 = 0 mm, d550_d538 = 0 mm, d551_d539 = 0 mm, d552_d546 = 0 mm, d553_d548 = 0 mm
